# Autodesk Inventor assembly: 구동부_어셈블
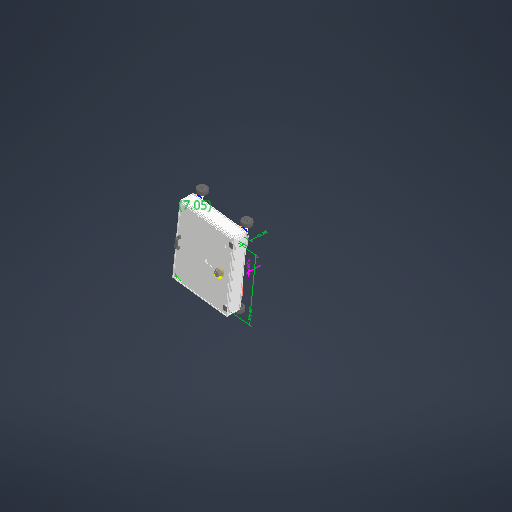
[picture p0: Inventor's stored thumbnail of the model, 512x512]
Saved by Autodesk Inventor 2026.2 (Build 302298010, 298A)
## iProperties
Created: 2026-06-08
Part Number: 구동부_어셈블
Document SubType Name: Assembly
Designer: dalbi
Author: dalbi
## Documents named in this file (17)
- C:\Users\User\Desktop\트리보 관련 자료\최종 설계 파일(조립시 참고할 파일)\구동부_어셈블.iam
- C:\Users\User\Desktop\트리보 관련 자료\최종 설계 파일(조립시 참고할 파일)\AL_Profile_20X20_640.ipt
- C:\Users\User\Desktop\트리보 관련 자료\최종 설계 파일(조립시 참고할 파일)\AL_Profile_20X20_80.ipt
- C:\Users\User\Desktop\트리보 관련 자료\최종 설계 파일(조립시 참고할 파일)\AL_Plate_Outer_600X460X2t_DriveTrain.ipt
- C:\Users\User\Desktop\트리보 관련 자료\최종 설계 파일(조립시 참고할 파일)\multiblock_12x12x14.ipt
- C:\Users\User\Desktop\트리보 관련 자료\최종 설계 파일(조립시 참고할 파일)\AL_Profile_20X20_460.ipt
- C:\Users\User\Desktop\트리보 관련 자료\최종 설계 파일(조립시 참고할 파일)\Motor_Tire_Assy.iam
- C:\Users\User\Desktop\트리보 관련 자료\최종 설계 파일(조립시 참고할 파일)\Motor_Cover_RH.ipt
- C:\Users\User\Desktop\트리보 관련 자료\최종 설계 파일(조립시 참고할 파일)\Acyril_Plate_Outer_460X80X5t.ipt
- C:\Users\User\Desktop\트리보 관련 자료\최종 설계 파일(조립시 참고할 파일)\Acryril_Plate_Outer_600X80X5t.ipt
- C:\Users\User\Desktop\트리보 관련 자료\최종 설계 파일(조립시 참고할 파일)\Acryil_door_600x460x2t.iam
- C:\Users\User\Desktop\트리보 관련 자료\최종 설계 파일(조립시 참고할 파일)\Door_Stopper.ipt
- C:\Users\User\Desktop\트리보 관련 자료\최종 설계 파일(조립시 참고할 파일)\Door_Stopper_2.ipt
- C:\Users\User\Desktop\트리보 관련 자료\최종 설계 파일(조립시 참고할 파일)\Acryril_Plate_Outer_600X80X5t_ChargeHole.ipt
- C:\Users\User\Desktop\트리보 관련 자료\최종 설계 파일(조립시 참고할 파일)\Motor_Cover_LH_V3.ipt
- C:\Users\User\Desktop\트리보 관련 자료\최종 설계 파일(조립시 참고할 파일)\Motor_Cover_RH_V3.ipt
- C:\Users\User\Desktop\트리보 관련 자료\최종 설계 파일(조립시 참고할 파일)\AL_Profile_20X20_600.ipt
## Components (53 placed, 16 different names)
1. AL_Profile_20X20_640:1 — 플러쉬:14, 메이트:7, 플러쉬:16, 플러쉬:21, 플러쉬:22, 플러쉬:36, 메이트:102, 플러쉬:110, 메이트:129
2. AL_Profile_20X20_640:2 — 플러쉬:17, 플러쉬:18, 플러쉬:19, 플러쉬:20, 메이트:46, 플러쉬:31, 플러쉬:32, 메이트:47, 플러쉬:33, 플러쉬:34, 메이트:58, 플러쉬:66, 메이트:86, 플러쉬:67, 메이트:87, 메이트:124, 메이트:126, 메이트:127, 메이트:130, 플러쉬:118, 메이트:134
3. AL_Profile_20X20_640:3 — 플러쉬:14, 메이트:7, 메이트:8, 플러쉬:15, 메이트:11, 메이트:14, 플러쉬:24, 메이트:32, 메이트:41, 플러쉬:27, 플러쉬:28, 메이트:44, 플러쉬:35, 플러쉬:108, 메이트:123, 메이트:137, 플러쉬:120, 메이트:139, 플러쉬:121, 플러쉬:122, 플러쉬:125, 메이트:146
4. AL_Profile_20X20_640:4 — 메이트:9, 메이트:10, 메이트:13, 메이트:35, 메이트:40, 플러쉬:25, 플러쉬:26, 메이트:45, 플러쉬:29, 플러쉬:30, 메이트:50, 메이트:54, 메이트:56, 플러쉬:58, 플러쉬:59, 메이트:80, 메이트:81, 플러쉬:64, 메이트:83, 플러쉬:65, 메이트:135, 플러쉬:119, 플러쉬:123, 플러쉬:124, 메이트:141, 플러쉬:126, 메이트:145
5. AL_Profile_20X20_80:1 — 메이트:8, 플러쉬:15, 플러쉬:16, 메이트:103, 메이트:110, 메이트:113
6. AL_Profile_20X20_80:2 — 메이트:9, 플러쉬:17, 플러쉬:18, 메이트:56, 플러쉬:58, 플러쉬:59, 메이트:58, 메이트:82, 메이트:85
7. AL_Profile_20X20_80:3 — 메이트:11, 플러쉬:21, 플러쉬:22, 플러쉬:35, 플러쉬:36, 메이트:94, 메이트:95, 메이트:101, 플러쉬:107, 메이트:122
8. AL_Profile_20X20_80:4 — 메이트:10, 플러쉬:19, 플러쉬:20, 메이트:84, 메이트:88, 메이트:89, 메이트:91, 메이트:116, 메이트:133
9. multiblock_12x12x14:1 — 메이트:13, 메이트:55, 플러쉬:56
10. multiblock_12x12x14:2 — 메이트:14, 플러쉬:24, 메이트:57
11. multiblock_12x12x14:3 — 메이트:53, 플러쉬:55, 메이트:54
12. multiblock_12x12x14:4 — 플러쉬:38, 메이트:49, 메이트:50
13. multiblock_12x12x14:5 — 메이트:32, 플러쉬:37, 메이트:48, 메이트:52
14. multiblock_12x12x14:6 — 메이트:35, 메이트:42, 메이트:51
15. AL_Profile_20X20_460:1 — 메이트:40, 플러쉬:25, 플러쉬:26, 메이트:41, 플러쉬:27, 플러쉬:28, 메이트:43, 메이트:53, 플러쉬:55, 메이트:55, 플러쉬:56, 메이트:57, 메이트:60, 메이트:69, 메이트:78, 메이트:79, 메이트:143
16. AL_Profile_20X20_460:2 — 메이트:45, 플러쉬:29, 플러쉬:30, 플러쉬:37, 메이트:48, 플러쉬:38, 메이트:49, 메이트:51, 메이트:68, 메이트:70, 메이트:73, 메이트:74, 플러쉬:69, 메이트:92, 메이트:96, 플러쉬:71, 메이트:117
17. AL_Profile_20X20_460:3 — 메이트:46, 플러쉬:31, 플러쉬:32, 플러쉬:68, 메이트:90, 메이트:93, 플러쉬:70, 메이트:128, 메이트:131
18. AL_Profile_20X20_460:4 — 메이트:47, 플러쉬:33, 플러쉬:34, 메이트:109, 플러쉬:116, 플러쉬:117, 메이트:111, 메이트:114, 메이트:125
19. AL_Plate_Outer_600X460X2t_DriveTrain:1 — 메이트:42, 메이트:43, 메이트:44, 메이트:52, 메이트:144
20. Motor_Tire_Assy:4 [sub-assembly] — 메이트:60, 메이트:69, 메이트:138, 플러쉬:125
21. Motor_Tire_Assy:5 [sub-assembly] — 메이트:68, 메이트:70, 메이트:136, 플러쉬:123
22. Motor_Tire_Assy:7 [sub-assembly] — 메이트:73, 메이트:74, 플러쉬:122, 메이트:140
23. Motor_Tire_Assy:8 [sub-assembly] — 메이트:78, 메이트:79, 플러쉬:124, 메이트:142
24. Motor_Cover_RH:2 — 메이트:80
25. multiblock_12x12x14:7 — 플러쉬:67, 메이트:87, 메이트:88
26. multiblock_12x12x14:8 — 메이트:85, 플러쉬:66, 메이트:86
27. multiblock_12x12x14:9 — 메이트:83, 플러쉬:65, 메이트:84, 메이트:132
28. multiblock_12x12x14:10 — 메이트:81, 플러쉬:64, 메이트:82
29. multiblock_12x12x14:11 — 메이트:93, 메이트:94, 플러쉬:70
30. multiblock_12x12x14:12 — 메이트:89, 플러쉬:68, 메이트:90
31. multiblock_12x12x14:13 — 메이트:95, 메이트:96, 플러쉬:71, 메이트:115
32. multiblock_12x12x14:14 — 메이트:91, 플러쉬:69, 메이트:92
33. multiblock_12x12x14:15 — 메이트:100, 플러쉬:102, 플러쉬:104, 메이트:101, 메이트:102, 플러쉬:107
34. multiblock_12x12x14:16 — 메이트:99, 플러쉬:102, 플러쉬:105, 플러쉬:106, 플러쉬:109, 플러쉬:110, 메이트:103, 메이트:121
35. multiblock_12x12x14:17 — 메이트:100, 플러쉬:103, 플러쉬:104, 플러쉬:108
36. multiblock_12x12x14:18 — 메이트:99, 플러쉬:103, 플러쉬:105, 플러쉬:106, 플러쉬:109
37. multiblock_12x12x14:19 — 메이트:104, 플러쉬:111, 플러쉬:112, 메이트:108, 메이트:109, 메이트:110, 플러쉬:116
38. multiblock_12x12x14:20 — 플러쉬:113, 메이트:106, 플러쉬:114, 플러쉬:115, 메이트:107, 메이트:108, 플러쉬:117, 메이트:111
39. multiblock_12x12x14:21 — 메이트:104, 플러쉬:111, 플러쉬:112, 메이트:105
40. multiblock_12x12x14:22 — 메이트:105, 플러쉬:113, 메이트:106, 플러쉬:114, 플러쉬:115, 메이트:107, 메이트:112
41. Acyril_Plate_Outer_460X80X5t:1 — 메이트:112, 메이트:113, 메이트:114
42. Acryril_Plate_Outer_600X80X5t:1 — 메이트:121, 메이트:122, 메이트:123
43. Acyril_Plate_Outer_460X80X5t:2 — 메이트:115, 메이트:116, 메이트:117
44. Acryil_door_600x460x2t:1 [sub-assembly] — 메이트:129, 메이트:130, 메이트:131
45. Door_Stopper:1 — 메이트:124, 메이트:125, 메이트:126
46. Door_Stopper_2:1 — 메이트:127, 메이트:128, 플러쉬:118
47. Acryril_Plate_Outer_600X80X5t_ChargeHole:1 — 메이트:132, 메이트:133, 메이트:134
48. Motor_Cover_LH_V3:1 — 메이트:137, 플러쉬:120, 메이트:138
49. Motor_Cover_LH_V3:2 — 메이트:135, 플러쉬:119, 메이트:136
50. Motor_Cover_RH_V3:1 — 메이트:139, 플러쉬:121, 메이트:140
51. Motor_Cover_RH_V3:2 — 메이트:141, 플러쉬:126, 메이트:142
52. AL_Profile_20X20_600:1 — 플러쉬:127, 플러쉬:128, 메이트:146
53. AL_Profile_20X20_600:2 — 플러쉬:127, 플러쉬:128, 메이트:143, 메이트:144, 메이트:145
## Relationships (163: Mate 100, Flush 63)
- 플러쉬:14 [Flush]: AL_Profile_20X20_640:1 ↔ AL_Profile_20X20_640:3
- 메이트:7 [Mate] (80 mm): AL_Profile_20X20_640:1 ↔ AL_Profile_20X20_640:3
- 메이트:8 [Mate]: AL_Profile_20X20_640:3 ↔ AL_Profile_20X20_80:1
- 플러쉬:15 [Flush]: AL_Profile_20X20_640:3 ↔ AL_Profile_20X20_80:1
- 플러쉬:16 [Flush]: AL_Profile_20X20_640:1 ↔ AL_Profile_20X20_80:1
- 메이트:9 [Mate]: AL_Profile_20X20_640:4 ↔ AL_Profile_20X20_80:2
- 플러쉬:17 [Flush]: AL_Profile_20X20_640:2 ↔ AL_Profile_20X20_80:2
- 플러쉬:18 [Flush]: AL_Profile_20X20_640:2 ↔ AL_Profile_20X20_80:2
- 메이트:10 [Mate]: AL_Profile_20X20_640:4 ↔ AL_Profile_20X20_80:4
- 플러쉬:19 [Flush]: AL_Profile_20X20_640:2 ↔ AL_Profile_20X20_80:4
- 플러쉬:20 [Flush]: AL_Profile_20X20_640:2 ↔ AL_Profile_20X20_80:4
- 메이트:11 [Mate]: AL_Profile_20X20_640:3 ↔ AL_Profile_20X20_80:3
- 플러쉬:21 [Flush]: AL_Profile_20X20_640:1 ↔ AL_Profile_20X20_80:3
- 플러쉬:22 [Flush]: AL_Profile_20X20_640:1 ↔ AL_Profile_20X20_80:3
- 메이트:13 [Mate]: AL_Profile_20X20_640:4 ↔ multiblock_12x12x14:1
- 메이트:14 [Mate]: AL_Profile_20X20_640:3 ↔ multiblock_12x12x14:2
- 플러쉬:24 [Flush] (3 mm): AL_Profile_20X20_640:3 ↔ multiblock_12x12x14:2
- 메이트:32 [Mate]: AL_Profile_20X20_640:3 ↔ multiblock_12x12x14:5
- 메이트:35 [Mate]: AL_Profile_20X20_640:4 ↔ multiblock_12x12x14:6
- 메이트:40 [Mate]: AL_Profile_20X20_640:4 ↔ AL_Profile_20X20_460:1
- 플러쉬:25 [Flush]: AL_Profile_20X20_640:4 ↔ AL_Profile_20X20_460:1
- 플러쉬:26 [Flush]: AL_Profile_20X20_640:4 ↔ AL_Profile_20X20_460:1
- 메이트:41 [Mate]: AL_Profile_20X20_640:3 ↔ AL_Profile_20X20_460:1
- 플러쉬:27 [Flush]: AL_Profile_20X20_640:3 ↔ AL_Profile_20X20_460:1
- 플러쉬:28 [Flush]: AL_Profile_20X20_640:3 ↔ AL_Profile_20X20_460:1
- 메이트:42 [Mate]: multiblock_12x12x14:6 ↔ AL_Plate_Outer_600X460X2t_DriveTrain:1
- 메이트:43 [Mate]: AL_Profile_20X20_460:1 ↔ AL_Plate_Outer_600X460X2t_DriveTrain:1
- 메이트:44 [Mate]: AL_Profile_20X20_640:3 ↔ AL_Plate_Outer_600X460X2t_DriveTrain:1
- 메이트:45 [Mate]: AL_Profile_20X20_640:4 ↔ AL_Profile_20X20_460:2
- 플러쉬:29 [Flush]: AL_Profile_20X20_640:4 ↔ AL_Profile_20X20_460:2
- 플러쉬:30 [Flush]: AL_Profile_20X20_640:4 ↔ AL_Profile_20X20_460:2
- 메이트:46 [Mate]: AL_Profile_20X20_640:2 ↔ AL_Profile_20X20_460:3
- 플러쉬:31 [Flush]: AL_Profile_20X20_640:2 ↔ AL_Profile_20X20_460:3
- 플러쉬:32 [Flush]: AL_Profile_20X20_640:2 ↔ AL_Profile_20X20_460:3
- 메이트:47 [Mate]: AL_Profile_20X20_640:2 ↔ AL_Profile_20X20_460:4
- 플러쉬:33 [Flush]: AL_Profile_20X20_640:2 ↔ AL_Profile_20X20_460:4
- 플러쉬:34 [Flush]: AL_Profile_20X20_640:2 ↔ AL_Profile_20X20_460:4
- 플러쉬:35 [Flush]: AL_Profile_20X20_640:3 ↔ AL_Profile_20X20_80:3
- 플러쉬:36 [Flush]: AL_Profile_20X20_640:1 ↔ AL_Profile_20X20_80:3
- 플러쉬:37 [Flush] (3 mm): multiblock_12x12x14:5 ↔ AL_Profile_20X20_460:2
- 메이트:48 [Mate]: multiblock_12x12x14:5 ↔ AL_Profile_20X20_460:2
- 플러쉬:38 [Flush] (3 mm): multiblock_12x12x14:4 ↔ AL_Profile_20X20_460:2
- 메이트:49 [Mate]: multiblock_12x12x14:4 ↔ AL_Profile_20X20_460:2
- 메이트:50 [Mate] (224 mm): AL_Profile_20X20_640:4 ↔ multiblock_12x12x14:4
- 메이트:51 [Mate]: multiblock_12x12x14:6 ↔ AL_Profile_20X20_460:2
- 메이트:52 [Mate]: multiblock_12x12x14:5 ↔ AL_Plate_Outer_600X460X2t_DriveTrain:1
- 메이트:53 [Mate]: multiblock_12x12x14:3 ↔ AL_Profile_20X20_460:1
- 플러쉬:55 [Flush] (3 mm): multiblock_12x12x14:3 ↔ AL_Profile_20X20_460:1
- 메이트:54 [Mate] (224 mm): AL_Profile_20X20_640:4 ↔ multiblock_12x12x14:3
- 메이트:55 [Mate]: multiblock_12x12x14:1 ↔ AL_Profile_20X20_460:1
- 플러쉬:56 [Flush] (3 mm): multiblock_12x12x14:1 ↔ AL_Profile_20X20_460:1
- 메이트:56 [Mate]: AL_Profile_20X20_640:4 ↔ AL_Profile_20X20_80:2
- 플러쉬:58 [Flush]: AL_Profile_20X20_640:4 ↔ AL_Profile_20X20_80:2
- 플러쉬:59 [Flush]: AL_Profile_20X20_640:4 ↔ AL_Profile_20X20_80:2
- 메이트:57 [Mate]: multiblock_12x12x14:2 ↔ AL_Profile_20X20_460:1
- 메이트:58 [Mate]: AL_Profile_20X20_640:2 ↔ AL_Profile_20X20_80:2
- 메이트:60 [Mate]: AL_Profile_20X20_460:1 ↔ Motor_Tire_Assy:4
- 메이트:68 [Mate]: AL_Profile_20X20_460:2 ↔ Motor_Tire_Assy:5
- 메이트:69 [Mate]: AL_Profile_20X20_460:1 ↔ Motor_Tire_Assy:4
- 메이트:70 [Mate]: AL_Profile_20X20_460:2 ↔ Motor_Tire_Assy:5
- 메이트:73 [Mate]: AL_Profile_20X20_460:2 ↔ Motor_Tire_Assy:7
- 메이트:74 [Mate]: AL_Profile_20X20_460:2 ↔ Motor_Tire_Assy:7
- [Mate]: Motor_Tire_Assy:8 ↔ Motor_Cover_RH:2
- [Mate]: Motor_Tire_Assy:8 ↔ Motor_Cover_RH:2
- 메이트:78 [Mate]: AL_Profile_20X20_460:1 ↔ Motor_Tire_Assy:8
- 메이트:79 [Mate]: AL_Profile_20X20_460:1 ↔ Motor_Tire_Assy:8
- 메이트:80 [Mate]: AL_Profile_20X20_640:4 ↔ Motor_Cover_RH:2
- 메이트:81 [Mate]: AL_Profile_20X20_640:4 ↔ multiblock_12x12x14:10
- 플러쉬:64 [Flush] (3 mm): AL_Profile_20X20_640:4 ↔ multiblock_12x12x14:10
- 메이트:82 [Mate]: AL_Profile_20X20_80:2 ↔ multiblock_12x12x14:10
- 메이트:83 [Mate]: AL_Profile_20X20_640:4 ↔ multiblock_12x12x14:9
- 플러쉬:65 [Flush] (3 mm): AL_Profile_20X20_640:4 ↔ multiblock_12x12x14:9
- 메이트:84 [Mate]: AL_Profile_20X20_80:4 ↔ multiblock_12x12x14:9
- 메이트:85 [Mate]: AL_Profile_20X20_80:2 ↔ multiblock_12x12x14:8
- 플러쉬:66 [Flush] (3 mm): AL_Profile_20X20_640:2 ↔ multiblock_12x12x14:8
- 메이트:86 [Mate]: AL_Profile_20X20_640:2 ↔ multiblock_12x12x14:8
- 플러쉬:67 [Flush] (3 mm): AL_Profile_20X20_640:2 ↔ multiblock_12x12x14:7
- 메이트:87 [Mate]: AL_Profile_20X20_640:2 ↔ multiblock_12x12x14:7
- 메이트:88 [Mate]: AL_Profile_20X20_80:4 ↔ multiblock_12x12x14:7
- 메이트:89 [Mate]: AL_Profile_20X20_80:4 ↔ multiblock_12x12x14:12
- 플러쉬:68 [Flush] (3 mm): AL_Profile_20X20_460:3 ↔ multiblock_12x12x14:12
- 메이트:90 [Mate]: AL_Profile_20X20_460:3 ↔ multiblock_12x12x14:12
- 메이트:91 [Mate]: AL_Profile_20X20_80:4 ↔ multiblock_12x12x14:14
- 플러쉬:69 [Flush] (3 mm): AL_Profile_20X20_460:2 ↔ multiblock_12x12x14:14
- 메이트:92 [Mate]: AL_Profile_20X20_460:2 ↔ multiblock_12x12x14:14
- 메이트:93 [Mate]: AL_Profile_20X20_460:3 ↔ multiblock_12x12x14:11
- 메이트:94 [Mate]: AL_Profile_20X20_80:3 ↔ multiblock_12x12x14:11
- 플러쉬:70 [Flush] (3 mm): AL_Profile_20X20_460:3 ↔ multiblock_12x12x14:11
- 메이트:95 [Mate]: AL_Profile_20X20_80:3 ↔ multiblock_12x12x14:13
- 메이트:96 [Mate]: AL_Profile_20X20_460:2 ↔ multiblock_12x12x14:13
- 플러쉬:71 [Flush] (3 mm): AL_Profile_20X20_460:2 ↔ multiblock_12x12x14:13
- 메이트:99 [Mate] (56 mm): multiblock_12x12x14:16 ↔ multiblock_12x12x14:18
- 메이트:100 [Mate] (56 mm): multiblock_12x12x14:15 ↔ multiblock_12x12x14:17
- 플러쉬:102 [Flush]: multiblock_12x12x14:15 ↔ multiblock_12x12x14:16
- 플러쉬:103 [Flush]: multiblock_12x12x14:17 ↔ multiblock_12x12x14:18
- 플러쉬:104 [Flush]: multiblock_12x12x14:15 ↔ multiblock_12x12x14:17
- 플러쉬:105 [Flush]: multiblock_12x12x14:16 ↔ multiblock_12x12x14:18
- 플러쉬:106 [Flush]: multiblock_12x12x14:16 ↔ multiblock_12x12x14:18
- 메이트:101 [Mate]: AL_Profile_20X20_80:3 ↔ multiblock_12x12x14:15
- 메이트:102 [Mate]: AL_Profile_20X20_640:1 ↔ multiblock_12x12x14:15
- 플러쉬:107 [Flush] (3 mm): AL_Profile_20X20_80:3 ↔ multiblock_12x12x14:15
- 플러쉬:108 [Flush] (3 mm): AL_Profile_20X20_640:3 ↔ multiblock_12x12x14:17
- 플러쉬:109 [Flush]: multiblock_12x12x14:16 ↔ multiblock_12x12x14:18
- 플러쉬:110 [Flush] (3 mm): AL_Profile_20X20_640:1 ↔ multiblock_12x12x14:16
- 메이트:103 [Mate]: AL_Profile_20X20_80:1 ↔ multiblock_12x12x14:16
- 메이트:104 [Mate] (56 mm): multiblock_12x12x14:19 ↔ multiblock_12x12x14:21
- 플러쉬:111 [Flush]: multiblock_12x12x14:19 ↔ multiblock_12x12x14:21
- 플러쉬:112 [Flush]: multiblock_12x12x14:19 ↔ multiblock_12x12x14:21
- 메이트:105 [Mate] (436 mm): multiblock_12x12x14:21 ↔ multiblock_12x12x14:22
- 플러쉬:113 [Flush]: multiblock_12x12x14:20 ↔ multiblock_12x12x14:22
- 메이트:106 [Mate] (56 mm): multiblock_12x12x14:20 ↔ multiblock_12x12x14:22
- 플러쉬:114 [Flush]: multiblock_12x12x14:20 ↔ multiblock_12x12x14:22
- 플러쉬:115 [Flush]: multiblock_12x12x14:20 ↔ multiblock_12x12x14:22
- 메이트:107 [Mate] (56 mm): multiblock_12x12x14:20 ↔ multiblock_12x12x14:22
- 메이트:108 [Mate] (436 mm): multiblock_12x12x14:19 ↔ multiblock_12x12x14:20
- 메이트:109 [Mate]: AL_Profile_20X20_460:4 ↔ multiblock_12x12x14:19
- 메이트:110 [Mate]: AL_Profile_20X20_80:1 ↔ multiblock_12x12x14:19
- 플러쉬:116 [Flush] (3 mm): AL_Profile_20X20_460:4 ↔ multiblock_12x12x14:19
- 플러쉬:117 [Flush] (3 mm): AL_Profile_20X20_460:4 ↔ multiblock_12x12x14:20
- 메이트:111 [Mate]: AL_Profile_20X20_460:4 ↔ multiblock_12x12x14:20
- 메이트:112 [Mate]: multiblock_12x12x14:22 ↔ Acyril_Plate_Outer_460X80X5t:1
- 메이트:113 [Mate]: AL_Profile_20X20_80:1 ↔ Acyril_Plate_Outer_460X80X5t:1
- 메이트:114 [Mate]: AL_Profile_20X20_460:4 ↔ Acyril_Plate_Outer_460X80X5t:1
- 메이트:115 [Mate]: multiblock_12x12x14:13 ↔ Acyril_Plate_Outer_460X80X5t:2
- 메이트:116 [Mate]: AL_Profile_20X20_80:4 ↔ Acyril_Plate_Outer_460X80X5t:2
- 메이트:117 [Mate]: AL_Profile_20X20_460:2 ↔ Acyril_Plate_Outer_460X80X5t:2
- 메이트:121 [Mate]: multiblock_12x12x14:16 ↔ Acryril_Plate_Outer_600X80X5t:1
- 메이트:122 [Mate]: AL_Profile_20X20_80:3 ↔ Acryril_Plate_Outer_600X80X5t:1
- 메이트:123 [Mate]: AL_Profile_20X20_640:3 ↔ Acryril_Plate_Outer_600X80X5t:1
- 메이트:124 [Mate]: AL_Profile_20X20_640:2 ↔ Door_Stopper:1
- 메이트:125 [Mate]: AL_Profile_20X20_460:4 ↔ Door_Stopper:1
- 메이트:126 [Mate]: AL_Profile_20X20_640:2 ↔ Door_Stopper:1
- 메이트:127 [Mate]: AL_Profile_20X20_640:2 ↔ Door_Stopper_2:1
- 메이트:128 [Mate]: AL_Profile_20X20_460:3 ↔ Door_Stopper_2:1
- 메이트:129 [Mate]: AL_Profile_20X20_640:1 ↔ Acryil_door_600x460x2t:1
- 메이트:130 [Mate]: AL_Profile_20X20_640:2 ↔ Acryil_door_600x460x2t:1
- 메이트:131 [Mate]: AL_Profile_20X20_460:3 ↔ Acryil_door_600x460x2t:1
- 플러쉬:118 [Flush] (20 mm): AL_Profile_20X20_640:2 ↔ Door_Stopper_2:1
- 메이트:132 [Mate]: multiblock_12x12x14:9 ↔ Acryril_Plate_Outer_600X80X5t_ChargeHole:1
- 메이트:133 [Mate]: AL_Profile_20X20_80:4 ↔ Acryril_Plate_Outer_600X80X5t_ChargeHole:1
- 메이트:134 [Mate]: AL_Profile_20X20_640:2 ↔ Acryril_Plate_Outer_600X80X5t_ChargeHole:1
- 메이트:135 [Mate]: AL_Profile_20X20_640:4 ↔ Motor_Cover_LH_V3:2
- 플러쉬:119 [Flush] (1 mm): AL_Profile_20X20_640:4 ↔ Motor_Cover_LH_V3:2
- 메이트:136 [Mate] (3 mm): Motor_Tire_Assy:5 ↔ Motor_Cover_LH_V3:2
- 메이트:137 [Mate]: AL_Profile_20X20_640:3 ↔ Motor_Cover_LH_V3:1
- 플러쉬:120 [Flush] (1 mm): AL_Profile_20X20_640:3 ↔ Motor_Cover_LH_V3:1
- 메이트:138 [Mate] (2 mm): Motor_Tire_Assy:4 ↔ Motor_Cover_LH_V3:1
- 메이트:139 [Mate]: AL_Profile_20X20_640:3 ↔ Motor_Cover_RH_V3:1
- 플러쉬:121 [Flush] (1 mm): AL_Profile_20X20_640:3 ↔ Motor_Cover_RH_V3:1
- 플러쉬:122 [Flush] (22 mm): AL_Profile_20X20_640:3 ↔ Motor_Tire_Assy:7
- 플러쉬:123 [Flush] (22 mm): AL_Profile_20X20_640:4 ↔ Motor_Tire_Assy:5
- 플러쉬:124 [Flush] (22 mm): AL_Profile_20X20_640:4 ↔ Motor_Tire_Assy:8
- 플러쉬:125 [Flush] (22 mm): AL_Profile_20X20_640:3 ↔ Motor_Tire_Assy:4
- 메이트:140 [Mate] (2 mm): Motor_Tire_Assy:7 ↔ Motor_Cover_RH_V3:1
- 메이트:141 [Mate]: AL_Profile_20X20_640:4 ↔ Motor_Cover_RH_V3:2
- 플러쉬:126 [Flush] (1 mm): AL_Profile_20X20_640:4 ↔ Motor_Cover_RH_V3:2
- 메이트:142 [Mate] (2 mm): Motor_Tire_Assy:8 ↔ Motor_Cover_RH_V3:2
- 플러쉬:127 [Flush]: AL_Profile_20X20_600:1 ↔ AL_Profile_20X20_600:2
- 플러쉬:128 [Flush]: AL_Profile_20X20_600:1 ↔ AL_Profile_20X20_600:2
- 메이트:143 [Mate]: AL_Profile_20X20_460:1 ↔ AL_Profile_20X20_600:2
- 메이트:144 [Mate]: AL_Plate_Outer_600X460X2t_DriveTrain:1 ↔ AL_Profile_20X20_600:2
- 메이트:145 [Mate] (150 mm): AL_Profile_20X20_640:4 ↔ AL_Profile_20X20_600:2
- 메이트:146 [Mate] (150 mm): AL_Profile_20X20_640:3 ↔ AL_Profile_20X20_600:1
## Named parameters: d130_d124 = 0 mm, d131_d125 = 0 mm
